# Autodesk Inventor assembly: intake1.1
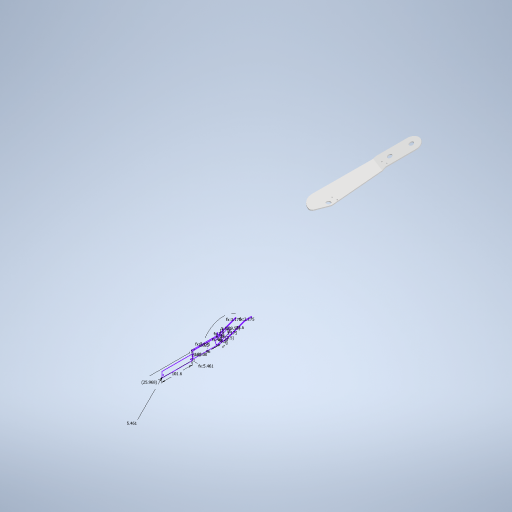
[picture p0: Inventor's stored thumbnail of the model, 512x512]
Saved by Autodesk Inventor 2023 (Build 270158000, 158)
## iProperties
Created: 2022-09-11
Part Number: intake1.1
Document SubType Name: Assembly
Designer: deli
Author: deli
## Documents named in this file (14)
- C:\Users\deli\OneDrive - Eastside Preparatory School\FTC\8103-power-play\CAD\intake1.1.iam
- C:\Users\deli\OneDrive - Eastside Preparatory School\FTC\8103-power-play\CAD\FTC-parts\am-4801_Blue am-4801_Red Cone REV2.ipt
- C:\Users\deli\OneDrive - Eastside Preparatory School\FTC\8103-power-play\CAD\Field Mat.ipt
- C:\Users\deli\OneDrive - Eastside Preparatory School\FTC\8103-power-play\CAD\FTC-parts\goBILDA\1611-0514-4008.ipt
- C:\Users\deli\OneDrive - Eastside Preparatory School\FTC\8103-power-play\CAD\FTC-parts\goBILDA\3613-4008-0048.ipt
- C:\Users\deli\OneDrive - Eastside Preparatory School\FTC\8103-power-play\CAD\FTC-parts\goBILDA\2801-0004-0011.ipt
- C:\Users\deli\OneDrive - Eastside Preparatory School\FTC\8103-power-play\CAD\FTC-parts\goBILDA\2802-0004-0010.ipt
- C:\Users\deli\OneDrive - Eastside Preparatory School\FTC\8103-power-play\CAD\FTC-parts\goBILDA\3613-0014-0096.ipt
- C:\Users\deli\OneDrive - Eastside Preparatory School\FTC\8103-power-play\CAD\FTC-parts\goBILDA\1309-0016-4008 assembly.ipt
- C:\Users\deli\OneDrive - Eastside Preparatory School\FTC\8103-power-play\CAD\FTC-parts\goBILDA\1522-0010-0040.ipt
- C:\Users\deli\OneDrive - Eastside Preparatory School\FTC\8103-power-play\CAD\IntakeHolder1.1.ipt
- C:\Users\deli\OneDrive - Eastside Preparatory School\FTC\8103-power-play\CAD\FTC-parts\goBILDA\1106-0002-0016.ipt
- C:\Users\deli\OneDrive - Eastside Preparatory School\FTC\8103-power-play\CAD\FTC-parts\goBILDA\3408-0001-0001 assembly.ipt
- C:\Users\deli\OneDrive - Eastside Preparatory School\FTC\8103-power-play\CAD\FTC-parts\goBILDA\3400-0014-0032.ipt
## Components (26 placed, 13 different names)
1. am-4801_Blue am-4801_Red Cone REV2:1 — Mate:1
2. Field Mat:1 — Mate:1, Mate:79, Angle:1
3. 1611-0514-4008:1 — Mate:66, Mate:67, Mate:84, Mate:85
4. 1611-0514-4008:4 — Mate:70, Mate:71, Mate:82, Mate:83
5. 3613-4008-0048:1 — Mate:26, Mate:27, Mate:56, Mate:57
6. 3613-4008-0048:2 — Mate:28, Mate:29, Mate:54, Mate:55, Mate:71
7. 2801-0004-0011:2 — Mate:26, Mate:27, Mate:68, Mate:69
8. 2801-0004-0011:3 — Mate:28, Mate:29, Mate:36, Mate:37
9. 2802-0004-0010:7 — Mate:36, Mate:37
10. 2802-0004-0010:8 — Mate:68, Mate:69
11. 1611-0514-4008:5 — Mate:80, Mate:81, Mate:88, Mate:89, Mate:107, Mate:108
12. 3613-0014-0096:1 — Mate:47, Mate:48, Mate:49, Mate:79
13. 1309-0016-4008 assembly:1 — Mate:47, Mate:48, Mate:49, Mate:86, Mate:87
14. 1522-0010-0040:1 — Mate:54, Mate:55, Mate:70
15. 1522-0010-0040:2 — Mate:56, Mate:57, Mate:66, Mate:67
16. IntakeHolder1.1:1 — Angle:1, Mate:80, Mate:81, Mate:82, Mate:83, Mate:84, Mate:85, Mate:90, Mate:91, Mate:92, Mate:93, Mate:95, Mate:96, Mate:97, Mate:98
17. 1522-0010-0040:5 — Mate:86, Mate:87, Mate:88, Mate:89
18. 1106-0002-0016:1 — Mate:90, Mate:91, Flush:1, Mate:103, Mate:104, Flush:5
19. 1106-0002-0016:2 — Mate:92, Mate:93, Flush:1, Mate:101, Mate:102, Flush:3
20. 1106-0002-0016:3 — Mate:96, Mate:98, Flush:2, Mate:99, Mate:100, Flush:4
21. 1106-0002-0016:4 — Mate:95, Mate:97, Flush:2, Mate:105, Mate:106, Flush:6
22. 3408-0001-0001 assembly:1 — Mate:101, Mate:102, Flush:3
23. 3408-0001-0001 assembly:2 — Mate:99, Mate:100, Flush:4
24. 3408-0001-0001 assembly:3 — Mate:105, Mate:106, Flush:6
25. 3408-0001-0001 assembly:4 — Mate:103, Mate:104, Flush:5
26. 3400-0014-0032:1 — Mate:107, Mate:108
## Relationships (56: Mate 49, Flush 6, Angle 1)
- Mate:1 (5.461 mm): am-4801_Blue am-4801_Red Cone REV2:1 ↔ Field Mat:1
- Mate:26: 3613-4008-0048:1 ↔ 2801-0004-0011:2
- Mate:27: 3613-4008-0048:1 ↔ 2801-0004-0011:2
- Mate:28: 3613-4008-0048:2 ↔ 2801-0004-0011:3
- Mate:29: 3613-4008-0048:2 ↔ 2801-0004-0011:3
- Mate:36: 2801-0004-0011:3 ↔ 2802-0004-0010:7
- Mate:37: 2801-0004-0011:3 ↔ 2802-0004-0010:7
- Mate:47: 3613-0014-0096:1 ↔ 1309-0016-4008 assembly:1
- Mate:48: 3613-0014-0096:1 ↔ 1309-0016-4008 assembly:1
- Mate:49: 3613-0014-0096:1 ↔ 1309-0016-4008 assembly:1
- Mate:54: 3613-4008-0048:2 ↔ 1522-0010-0040:1
- Mate:55: 3613-4008-0048:2 ↔ 1522-0010-0040:1
- Mate:56: 3613-4008-0048:1 ↔ 1522-0010-0040:2
- Mate:57: 3613-4008-0048:1 ↔ 1522-0010-0040:2
- Mate:66: 1611-0514-4008:1 ↔ 1522-0010-0040:2
- Mate:67: 1611-0514-4008:1 ↔ 1522-0010-0040:2
- Mate:68: 2801-0004-0011:2 ↔ 2802-0004-0010:8
- Mate:69: 2801-0004-0011:2 ↔ 2802-0004-0010:8
- Mate:70: 1611-0514-4008:4 ↔ 1522-0010-0040:1
- Mate:71: 1611-0514-4008:4 ↔ 3613-4008-0048:2
- Mate:79 (4 mm): Field Mat:1 ↔ 3613-0014-0096:1
- Angle:1 (0 deg): Field Mat:1 ↔ IntakeHolder1.1:1
- Mate:80: 1611-0514-4008:5 ↔ IntakeHolder1.1:1
- Mate:81: 1611-0514-4008:5 ↔ IntakeHolder1.1:1
- Mate:82: 1611-0514-4008:4 ↔ IntakeHolder1.1:1
- Mate:83: 1611-0514-4008:4 ↔ IntakeHolder1.1:1
- Mate:84: 1611-0514-4008:1 ↔ IntakeHolder1.1:1
- Mate:85: 1611-0514-4008:1 ↔ IntakeHolder1.1:1
- Mate:86: 1309-0016-4008 assembly:1 ↔ 1522-0010-0040:5
- Mate:87: 1309-0016-4008 assembly:1 ↔ 1522-0010-0040:5
- Mate:88: 1611-0514-4008:5 ↔ 1522-0010-0040:5
- Mate:89: 1611-0514-4008:5 ↔ 1522-0010-0040:5
- Mate:90: IntakeHolder1.1:1 ↔ 1106-0002-0016:1
- Mate:91: IntakeHolder1.1:1 ↔ 1106-0002-0016:1
- Mate:92: IntakeHolder1.1:1 ↔ 1106-0002-0016:2
- Mate:93: IntakeHolder1.1:1 ↔ 1106-0002-0016:2
- Mate:95: IntakeHolder1.1:1 ↔ 1106-0002-0016:4
- Mate:96: IntakeHolder1.1:1 ↔ 1106-0002-0016:3
- Mate:97: IntakeHolder1.1:1 ↔ 1106-0002-0016:4
- Mate:98: IntakeHolder1.1:1 ↔ 1106-0002-0016:3
- Flush:1: 1106-0002-0016:1 ↔ 1106-0002-0016:2
- Flush:2: 1106-0002-0016:3 ↔ 1106-0002-0016:4
- Mate:99: 1106-0002-0016:3 ↔ 3408-0001-0001 assembly:2
- Mate:100: 1106-0002-0016:3 ↔ 3408-0001-0001 assembly:2
- Mate:101: 1106-0002-0016:2 ↔ 3408-0001-0001 assembly:1
- Mate:102: 1106-0002-0016:2 ↔ 3408-0001-0001 assembly:1
- Flush:3: 1106-0002-0016:2 ↔ 3408-0001-0001 assembly:1
- Flush:4: 1106-0002-0016:3 ↔ 3408-0001-0001 assembly:2
- Mate:103: 1106-0002-0016:1 ↔ 3408-0001-0001 assembly:4
- Mate:104: 1106-0002-0016:1 ↔ 3408-0001-0001 assembly:4
- Flush:5: 1106-0002-0016:1 ↔ 3408-0001-0001 assembly:4
- Mate:105: 1106-0002-0016:4 ↔ 3408-0001-0001 assembly:3
- Mate:106: 1106-0002-0016:4 ↔ 3408-0001-0001 assembly:3
- Flush:6: 1106-0002-0016:4 ↔ 3408-0001-0001 assembly:3
- Mate:107: 1611-0514-4008:5 ↔ 3400-0014-0032:1
- Mate:108: 1611-0514-4008:5 ↔ 3400-0014-0032:1
